# Autodesk Inventor assembly: Universal Shaft Angle
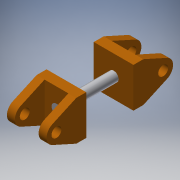
[picture p0: Inventor's stored thumbnail of the model, 180x180]
Saved by Autodesk Inventor 2016 (Build 200138000, 138)
## iProperties
Created: 2014-03-12
Part Number: Universal Shaft Angle
Document SubType Name: Assembly
Designer: John
Author: John
## Documents named in this file (3)
- C:\File Storage\Autodesk\Inventor 2016 Projects\Ex_Files_Inventor_2016_EssT\Exercise Files\15_Using constraints to position parts\15_02\Universal Shaft Angle.iam
- C:\File Storage\Autodesk\Inventor 2016 Projects\Ex_Files_Inventor_2016_EssT\Exercise Files\15_Using constraints to position parts\15_02\Joint.ipt
- C:\File Storage\Autodesk\Inventor 2016 Projects\Ex_Files_Inventor_2016_EssT\Exercise Files\15_Using constraints to position parts\15_02\Connecting Rod.ipt
## Components (3 placed, 2 different names)
1. Joint:3 — Flush:1, Mate:1
2. Connecting Rod:1 — Flush:1, Mate:1, Flush:2, Mate:2
3. Joint:4 — Flush:2, Mate:2
## Relationships (4: Flush 2, Mate 2)
- Flush:1: Joint:3 ↔ Connecting Rod:1
- Mate:1: Joint:3 ↔ Connecting Rod:1
- Flush:2: Connecting Rod:1 ↔ Joint:4
- Mate:2: Connecting Rod:1 ↔ Joint:4
